# Autodesk Inventor assembly: soloactuador
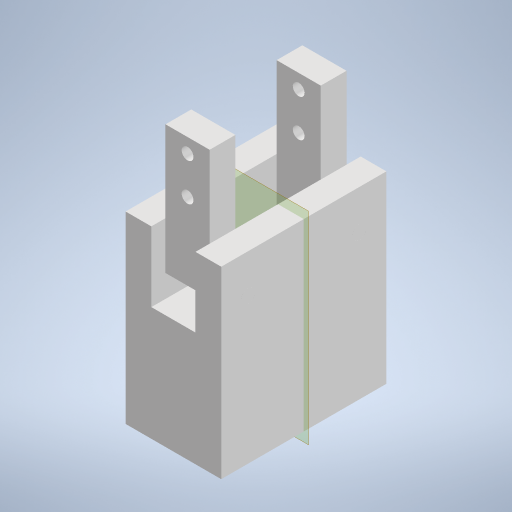
[picture p0: Inventor's stored thumbnail of the model, 512x512]
Saved by Autodesk Inventor 2024.3 (Build 283343000, 343)
## iProperties
Created: 2025-07-09
Part Number: soloactuador
Document SubType Name: Assembly
Designer: user
Author: user
## Documents named in this file (6)
- C:\Users\user\Desktop\Unal\Robotica\proyecto\garra neumatica\soloactuador.iam
- C:\Users\user\Desktop\Unal\Robotica\proyecto\garra neumatica\housing.ipt
- C:\Users\user\Desktop\Unal\Robotica\proyecto\garra neumatica\eje.ipt
- C:\Users\user\Desktop\Unal\Robotica\proyecto\garra neumatica\dedos.ipt
- C:\Users\user\Desktop\Unal\Robotica\proyecto\garra neumatica\eje_MIR1.ipt
- C:\Users\user\Desktop\Unal\Robotica\proyecto\garra neumatica\dedos_MIR1.ipt
## Components (5 placed, 5 different names)
1. housing:1 — Rigid:1, Rotational:1, Mate:1, Angle:1
2. eje:1 — Rigid:1
3. dedos:1 — Rotational:1
4. eje_MIR1:1
5. dedos_MIR1:1
## Relationships (4: WeldJoint 1, RevoluteJoint 1, Mate 1, Angle 1)
- Rigid:1 [WeldJoint]: housing:1 ↔ eje:1
- Rotational:1 [RevoluteJoint]: housing:1 ↔ dedos:1
- Mate:1: housing:1
- Angle:1 (0 deg): housing:1
